# Autodesk Inventor assembly: МД.001.200 - Редуктор планетарный
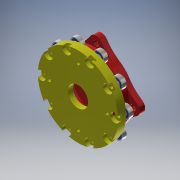
[picture p0: Inventor's stored thumbnail of the model, 180x180]
Saved by Autodesk Inventor 2019 (Build 230136000, 136)
## iProperties
Created: 2019-12-22
Part Number: МД.001.200 - Редуктор планетарный
Material: Типовые
Document SubType Name: Assembly
Designer: Петров Иван
Author: Петров Иван
## Documents named in this file (4)
- E:\IVAN\Ivan_desktop\GitHub\Arm_manip\hardware\МД.001.200 - Редуктор планетарный.iam
- E:\IVAN\Ivan_desktop\GitHub\Arm_manip\hardware\Standart_things\Подшипник 624Z.ipt
- E:\IVAN\Ivan_desktop\GitHub\Arm_manip\hardware\МД.001.202 - Корона.ipt
- E:\IVAN\Ivan_desktop\GitHub\Arm_manip\hardware\МД.001.201 - Основа.ipt
## Components (12 placed, 3 different names)
1. МД.001.201 - Основа:1 — Совмещение:1, Совмещение:2, Совмещение:3, Совмещение:4, Совмещение:5, Совмещение:6, Совмещение:7, Совмещение:8, Совмещение:9, Совмещение:10, Совмещение:11, Совмещение:12, Совмещение:13, Совмещение:14, Совмещение:15, Совмещение:16, Совмещение:17, Совмещение:18, Совмещение:19, Совмещение:20, Совмещение:22, Вставка:1
2. Подшипник 624Z:1 — Совмещение:1, Совмещение:2
3. Подшипник 624Z:2 — Совмещение:3, Совмещение:4
4. Подшипник 624Z:3 — Совмещение:5, Совмещение:6, Совмещение:21
5. Подшипник 624Z:4 — Совмещение:7, Совмещение:8, Касательность:3
6. Подшипник 624Z:5 — Совмещение:9, Совмещение:10
7. Подшипник 624Z:6 — Совмещение:11, Совмещение:12
8. Подшипник 624Z:7 — Совмещение:13, Совмещение:14
9. Подшипник 624Z:8 — Совмещение:15, Совмещение:16
10. Подшипник 624Z:9 — Совмещение:17, Совмещение:18, Касательность:2
11. Подшипник 624Z:10 — Совмещение:19, Совмещение:20, Касательность:1
12. МД.001.202 - Корона:1 — Касательность:1, Касательность:2, Касательность:3, Совмещение:21, Совмещение:22, Вставка:1
## Relationships (26: Mate 22, Tangent 3, Insert 1)
- Совмещение:1 [Mate]: МД.001.201 - Основа:1 ↔ Подшипник 624Z:1
- Совмещение:2 [Mate] (1 mm): МД.001.201 - Основа:1 ↔ Подшипник 624Z:1
- Совмещение:3 [Mate] (1 mm): МД.001.201 - Основа:1 ↔ Подшипник 624Z:2
- Совмещение:4 [Mate]: МД.001.201 - Основа:1 ↔ Подшипник 624Z:2
- Совмещение:5 [Mate] (1 mm): МД.001.201 - Основа:1 ↔ Подшипник 624Z:3
- Совмещение:6 [Mate]: МД.001.201 - Основа:1 ↔ Подшипник 624Z:3
- Совмещение:7 [Mate] (1 mm): МД.001.201 - Основа:1 ↔ Подшипник 624Z:4
- Совмещение:8 [Mate]: МД.001.201 - Основа:1 ↔ Подшипник 624Z:4
- Совмещение:9 [Mate] (1 mm): МД.001.201 - Основа:1 ↔ Подшипник 624Z:5
- Совмещение:10 [Mate]: МД.001.201 - Основа:1 ↔ Подшипник 624Z:5
- Совмещение:11 [Mate] (1 mm): МД.001.201 - Основа:1 ↔ Подшипник 624Z:6
- Совмещение:12 [Mate]: МД.001.201 - Основа:1 ↔ Подшипник 624Z:6
- Совмещение:13 [Mate] (1 mm): МД.001.201 - Основа:1 ↔ Подшипник 624Z:7
- Совмещение:14 [Mate]: МД.001.201 - Основа:1 ↔ Подшипник 624Z:7
- Совмещение:15 [Mate] (1 mm): МД.001.201 - Основа:1 ↔ Подшипник 624Z:8
- Совмещение:16 [Mate]: МД.001.201 - Основа:1 ↔ Подшипник 624Z:8
- Совмещение:17 [Mate] (1 mm): МД.001.201 - Основа:1 ↔ Подшипник 624Z:9
- Совмещение:18 [Mate]: МД.001.201 - Основа:1 ↔ Подшипник 624Z:9
- Совмещение:19 [Mate] (1 mm): МД.001.201 - Основа:1 ↔ Подшипник 624Z:10
- Совмещение:20 [Mate]: МД.001.201 - Основа:1 ↔ Подшипник 624Z:10
- Касательность:1 [Tangent]: Подшипник 624Z:10 ↔ МД.001.202 - Корона:1
- Касательность:2 [Tangent]: Подшипник 624Z:9 ↔ МД.001.202 - Корона:1
- Касательность:3 [Tangent]: Подшипник 624Z:4 ↔ МД.001.202 - Корона:1
- Совмещение:21 [Mate]: Подшипник 624Z:3 ↔ МД.001.202 - Корона:1
- Совмещение:22 [Mate]: МД.001.201 - Основа:1 ↔ МД.001.202 - Корона:1
- Вставка:1 [Insert] (-6 mm): МД.001.201 - Основа:1 ↔ МД.001.202 - Корона:1
